# Autodesk Inventor assembly: assembly first
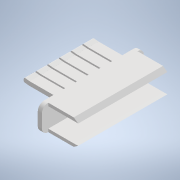
[picture p0: Inventor's stored thumbnail of the model, 180x180]
Saved by Autodesk Inventor 2020.2 (Build 242310000, 310)
## iProperties
Created: 2020-05-05
Part Number: assembly first
Document SubType Name: Assembly
Designer: Amaan Khalid
Author: Amaan Khalid
## Documents named in this file (3)
- C:\Users\Amaan Khalid\Desktop\my jumper cablehodler\assembly first.iam
- C:\Users\Amaan Khalid\Desktop\my jumper cablehodler\hook thing.ipt
- C:\Users\Amaan Khalid\Desktop\my jumper cablehodler\the whole thing.ipt
## Components (6 placed, 2 different names)
1. the whole thing:1 — Mate:1, Flush:1, Mate:2, Flush:2, Mate:3, Flush:3, Mate:4, Flush:4, Mate:5, Flush:5, Flush:6, Flush:7, Flush:8, Flush:9, Flush:10
2. hook thing:2 — Mate:4, Flush:4, Flush:9
3. hook thing:3 — Mate:3, Flush:3, Flush:8
4. hook thing:4 — Mate:1, Flush:1, Flush:6
5. hook thing:5 — Mate:2, Flush:2, Flush:7
6. hook thing:7 — Mate:5, Flush:5, Flush:10
## Relationships (15: Flush 10, Mate 5)
- Mate:1: the whole thing:1 ↔ hook thing:4
- Flush:1: the whole thing:1 ↔ hook thing:4
- Mate:2: the whole thing:1 ↔ hook thing:5
- Flush:2: the whole thing:1 ↔ hook thing:5
- Mate:3: the whole thing:1 ↔ hook thing:3
- Flush:3: the whole thing:1 ↔ hook thing:3
- Mate:4: the whole thing:1 ↔ hook thing:2
- Flush:4: the whole thing:1 ↔ hook thing:2
- Mate:5: the whole thing:1 ↔ hook thing:7
- Flush:5: the whole thing:1 ↔ hook thing:7
- Flush:6: the whole thing:1 ↔ hook thing:4
- Flush:7: the whole thing:1 ↔ hook thing:5
- Flush:8: the whole thing:1 ↔ hook thing:3
- Flush:9: the whole thing:1 ↔ hook thing:2
- Flush:10: the whole thing:1 ↔ hook thing:7
